# Autodesk Inventor assembly: PDRM25
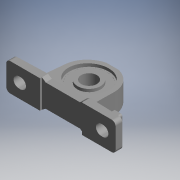
[picture p0: Inventor's stored thumbnail of the model, 180x180]
Saved by Autodesk Inventor 2017.3 (Build 213256000, 256)
## iProperties
Category: PARTsolutions
Company: MISUMI
Part Number: PDRM25
Catalog Web Link: www.cadenas.de
Description: PDRM-Ball Bearing Units - Pillow Casting Housing Type -
Vendor: MISUMI
Document SubType Name: Assembly
Designer: partserver
Manufacturer: MISUMI
Mass: 209.967 g
Surface Area: 416.706 cm^2
Volume: 209.967 cm^3
Density: 1 g/cm^3
Title: PDRM25
Author: Cadenas PARTsolutions
Comments: Ball Bearing Units - Pillow Casting Housing Type -
PSOL_IDENT_0: {$CADENAS_DATA\23d-libs\misumi\metric\12_bearing_holders\pdrm_asmtab.prj},164 {VTYP=3D},{STYP=ASSTAB
PSOL_IDENT_1: },{NB=PDRM25},{LINA=PDRM25},{NN=PDRM},{DATE=18.09.2019 02:29:27},{GEOMDATE=03.09.2019 09:06:38},{VER
PSOL_IDENT_2: SION=},{LINEID=10},{WBVAR=},{WBNUMERIC=}  {NB=PDRM25},{LINA=PDRM25},{KT=DUMMY},{PN=PDRM25},{TYPE=PDR
PSOL_IDENT_3: M},{MTH=Alloy Cast Iron Class No.30},{MTB=52100 Bearing Steel},{MTRS=Silicon Rubber},{MTSS=4137 Allo
PSOL_IDENT_4: y Steel},{PRECISION=JIS B 1558, JIS B 1559},{OT=-15 ~+100},{D=25},{JIS=UCP305},{H=45},{L=175},{L1=13
PSOL_IDENT_5: 2},{A=45},{DD1=20},{DD=17},{TT=16},{H1=84},{B=38},{S=15},{CRR=21.3},{COR=10.9},{M1=M6x0.75},{M1ALG=6
PSOL_IDENT_6: },{T=390},{ALC=1065},{MASS=1600},{HR1=39},{HR2=63},{HR3=58.335},{HR4=36.9},{HH1=11},{HH2=13},{HW2=55
PSOL_IDENT_7: },{HW3=67},{HW4=80.5},{HA1=2.186},{HW5=36.5},{HW6=29},{R1=3},{R2=15},{R3=6},{LEN1=82.5},{LEN2=15},{W=
PSOL_IDENT_8: 30},{BW=21},{GZ=5.0},{LS=8},{PPATH=pdrm/pdrm_asmtpl.prj}
NB: PDRM25
NN: PDRM
NT: Ball Bearing Units - Pillow Casting Housing Type -
NBSYN: $PN.
LINA: PDRM25
CATALOG: Misumi
PN: PDRM25
TYPE: PDRM
MTH: Alloy Cast Iron Class No.30
MTB: 52100 Bearing Steel
MTRS: Silicon Rubber
MTSS: 4137 Alloy Steel
PRECISION: JIS B 1558, JIS B 1559
OT: -15 ~+100
D: 25
JIS: UCP305
H: 45
L: 175
L1: 132
A: 45
DD1: 20
DD: 17
TT: 16
H1: 84
B: 38
S: 15
CRR: 21.3
COR: 10.9
M1: M6x0.75
T: 390
ALC: 1065
MASS: 1600
PPATH: pdrm/pdrm_asmtpl.prj
SUPPLIER: MISUMI
ARTICLENO: PDRM25
BOMINFO: PDRM25
CREATOR: CADENAS GmbH
## Documents named in this file (3)
- e:\temp\worker_13\temp\exporttempdir_2212_208_wOjDe\format_0\PDRM25.iam
- e:\temp\worker_13\temp\exporttempdir_2212_208_wOjDe\format_0\PDRM25_b.ipt
- e:\temp\worker_13\temp\exporttempdir_2212_208_wOjDe\format_0\SET-SCREW6-8.ipt
## Components (3 placed, 2 different names)
1. PDRM25_b:1 — cp1_XY@1 <-> CP_XY@2, cp1_Z@1 <-> CP_Z@2, cp1_YZ@1 <-> CP_YZ@2, cp2_XY@1 <-> CP_XY@3, cp2_Z@1 <-> CP_Z@3, cp2_YZ@1 <-> CP_YZ@3
2. SET-SCREW6-8:1 — cp1_XY@1 <-> CP_XY@2, cp1_Z@1 <-> CP_Z@2, cp1_YZ@1 <-> CP_YZ@2
3. SET-SCREW6-8:2 — cp2_XY@1 <-> CP_XY@3, cp2_Z@1 <-> CP_Z@3, cp2_YZ@1 <-> CP_YZ@3
## Relationships (6: Mate 4, Angle 2)
- cp1_XY@1 <-> CP_XY@2 [Mate]: PDRM25_b:1 ↔ SET-SCREW6-8:1
- cp1_Z@1 <-> CP_Z@2 [Mate]: PDRM25_b:1 ↔ SET-SCREW6-8:1
- cp1_YZ@1 <-> CP_YZ@2 [Angle] (0 deg): PDRM25_b:1 ↔ SET-SCREW6-8:1
- cp2_XY@1 <-> CP_XY@3 [Mate]: PDRM25_b:1 ↔ SET-SCREW6-8:2
- cp2_Z@1 <-> CP_Z@3 [Mate]: PDRM25_b:1 ↔ SET-SCREW6-8:2
- cp2_YZ@1 <-> CP_YZ@3 [Angle] (0 deg): PDRM25_b:1 ↔ SET-SCREW6-8:2
